# Autodesk Inventor assembly: Absorber IHF X-Gantry
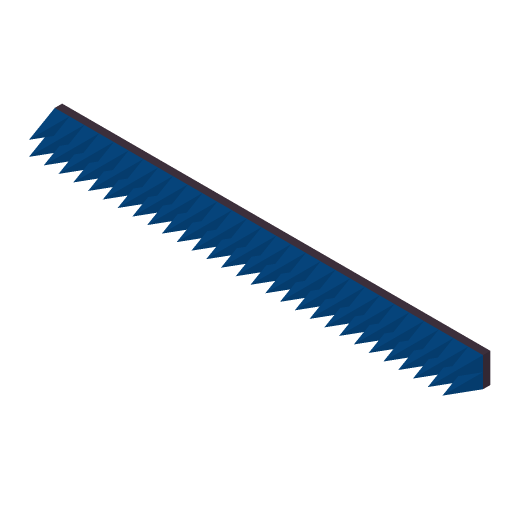
[picture p0: Inventor's stored thumbnail of the model, 512x512]
Saved by Autodesk Inventor 2023.2 (Build 272271000, 271)
## iProperties
Created: 2024-03-07
Part Number: Absorber IHF X-Gantry
Document SubType Name: Assembly
Designer: Nils Bade
Author: Nils Bade
## Documents named in this file (2)
- C:\Users\nilsb\Documents\Inventor\Projektarbeit-Bade\Enclosure\Absorber\Absorber IHF X-Gantry.iam
- C:\Users\nilsb\Documents\Inventor\Projektarbeit-Bade\Enclosure\Absorber\Absorber - IHF-Mini.ipt
## Components (58 placed, 1 different names)
1. Absorber - IHF-Mini:1
2. Absorber - IHF-Mini:2
3. Absorber - IHF-Mini:3
4. Absorber - IHF-Mini:4
5. Absorber - IHF-Mini:5
6. Absorber - IHF-Mini:6
7. Absorber - IHF-Mini:7
8. Absorber - IHF-Mini:8
9. Absorber - IHF-Mini:9
10. Absorber - IHF-Mini:10
11. Absorber - IHF-Mini:11
12. Absorber - IHF-Mini:12
13. Absorber - IHF-Mini:13
14. Absorber - IHF-Mini:14
15. Absorber - IHF-Mini:15
16. Absorber - IHF-Mini:16
17. Absorber - IHF-Mini:17
18. Absorber - IHF-Mini:18
19. Absorber - IHF-Mini:19
20. Absorber - IHF-Mini:20
21. Absorber - IHF-Mini:21
22. Absorber - IHF-Mini:22
23. Absorber - IHF-Mini:23
24. Absorber - IHF-Mini:24
25. Absorber - IHF-Mini:25
26. Absorber - IHF-Mini:26
27. Absorber - IHF-Mini:27
28. Absorber - IHF-Mini:28
29. Absorber - IHF-Mini:29
30. Absorber - IHF-Mini:30
31. Absorber - IHF-Mini:31
32. Absorber - IHF-Mini:32
33. Absorber - IHF-Mini:33
34. Absorber - IHF-Mini:34
35. Absorber - IHF-Mini:35
36. Absorber - IHF-Mini:36
37. Absorber - IHF-Mini:37
38. Absorber - IHF-Mini:38
39. Absorber - IHF-Mini:39
40. Absorber - IHF-Mini:40
41. Absorber - IHF-Mini:41
42. Absorber - IHF-Mini:42
43. Absorber - IHF-Mini:43
44. Absorber - IHF-Mini:44
45. Absorber - IHF-Mini:45
46. Absorber - IHF-Mini:46
47. Absorber - IHF-Mini:47
48. Absorber - IHF-Mini:48
49. Absorber - IHF-Mini:49
50. Absorber - IHF-Mini:50
51. Absorber - IHF-Mini:51
52. Absorber - IHF-Mini:52
53. Absorber - IHF-Mini:53
54. Absorber - IHF-Mini:54
55. Absorber - IHF-Mini:55
56. Absorber - IHF-Mini:56
57. Absorber - IHF-Mini:57
58. Absorber - IHF-Mini:58
## Component patterns: (58 elements, first: Absorber - IHF-Mini:1)
